# Autodesk Inventor assembly: obj2iam
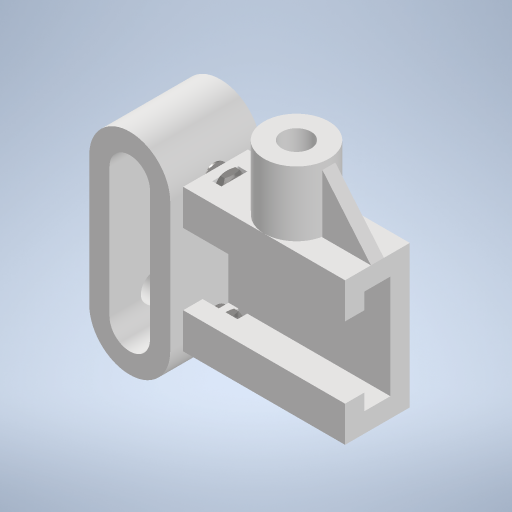
[picture p0: Inventor's stored thumbnail of the model, 512x512]
Saved by Autodesk Inventor 2023.2 (Build 272271030, 271C)
## iProperties
Created: 2023-02-25
Part Number: obj2iam
Document SubType Name: Assembly
Designer: Cris Pat
Author: Cris Pat
## Documents named in this file (7)
- C:\Users\Cris Pat\Desktop\U\Semestre 9\disenio e innovacion\CAD\obj2iam.iam
- C:\Users\Cris Pat\Desktop\U\Semestre 9\disenio e innovacion\CAD\cilindro_obj2.ipt
- C:\Users\Cris Pat\Desktop\U\Semestre 9\disenio e innovacion\CAD\cuerpo_obj2.ipt
- C:\Users\Cris Pat\Desktop\U\Semestre 9\disenio e innovacion\CAD\cabeza_obj2.ipt
- C:\Users\Cris Pat\Documents\Inventor\Content Center Files\R2023\en-US\DIN 84\DIN 84 - M5 x 12.ipt
- C:\Users\Cris Pat\Documents\Inventor\Content Center Files\R2023\en-US\DIN 84\DIN 84 - M5 x 14.ipt
- C:\Users\Cris Pat\Documents\Inventor\Content Center Files\R2023\en-US\DIN 439-2\DIN 439 - M5 x 0.8.ipt
## Components (9 placed, 6 different names)
1. cilindro_obj2:1 — Rotational:1, Rigid:1
2. cuerpo_obj2:1 — Rigid:1, Rotational:2, Rigid:2, Rotational:3, Rotational:4
3. cabeza_obj2:1 — Rigid:2, Rigid:3, Rigid:4
4. DIN 84 - replaced by DIN EN ISO 1207 M5 x 14:1 — Rotational:1
5. DIN 84 - replaced by DIN EN ISO 1207 M5 x 12:2 — Rigid:3
6. DIN 84 - replaced by DIN EN ISO 1207 M5 x 12:3 — Rigid:4
7. DIN 439-2 - replaced by DIN EN 24035/28675 M5:1 — Rotational:2
8. DIN 439-2 - replaced by DIN EN 24035/28675 M5:2 — Rotational:4
9. DIN 439-2 - replaced by DIN EN 24035/28675 M5:3 — Rotational:3
## Relationships (8: RevoluteJoint 4, WeldJoint 4)
- Rotational:1 [RevoluteJoint]: cilindro_obj2:1 ↔ DIN 84 - replaced by DIN EN ISO 1207 M5 x 14:1
- Rigid:1 [WeldJoint]: cilindro_obj2:1 ↔ cuerpo_obj2:1
- Rotational:2 [RevoluteJoint]: cuerpo_obj2:1 ↔ DIN 439-2 - replaced by DIN EN 24035/28675 M5:1
- Rigid:2 [WeldJoint]: cuerpo_obj2:1 ↔ cabeza_obj2:1
- Rigid:3 [WeldJoint]: cabeza_obj2:1 ↔ DIN 84 - replaced by DIN EN ISO 1207 M5 x 12:2
- Rigid:4 [WeldJoint]: cabeza_obj2:1 ↔ DIN 84 - replaced by DIN EN ISO 1207 M5 x 12:3
- Rotational:3 [RevoluteJoint]: cuerpo_obj2:1 ↔ DIN 439-2 - replaced by DIN EN 24035/28675 M5:3
- Rotational:4 [RevoluteJoint]: cuerpo_obj2:1 ↔ DIN 439-2 - replaced by DIN EN 24035/28675 M5:2
